# Autodesk Inventor assembly: A1-19027-400-06 Flange Comparison
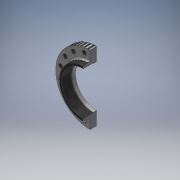
[picture p0: Inventor's stored thumbnail of the model, 180x180]
Saved by Autodesk Inventor 2017.3 (Build 213257000, 257)
## iProperties
Created: 2020-03-12
Part Number: A1-19027-400-06 Flange Comparison
Document SubType Name: Assembly
Designer: BEM
Author: BEM
## Documents named in this file (4)
- N:\A1 - Projects\A1-19\A1-19027--Syncrude Aurora HT2 spools - SP-237\A1-19027-400-06 Flange Comparison.iam
- N:\A1 - Projects\A1-19\A1-19027--Syncrude Aurora HT2 spools - SP-237\A1-19027-400-06 Alco flange - 12in CL300.ipt
- N:\Inventor\Content Center Files\R2017\en-US\ASME B16.5(10)\ASME B16.5 Flange Lapped - Class 300 12.ipt
- N:\Inventor\Content Center Files\R2017\en-US\ASME B16.5(41)\ASME B16.5 Flange Welding Neck - Class 300 12.ipt
## Components (3 placed, 3 different names)
1. A1-19027-400-06 Alco flange - 12in CL300:1 — Mate:1, Flush:1
2. ASME B16.5 Flange Lapped - Class 300 12:1 — Mate:1, Mate:2, Flush:2
3. ASME B16.5 Flange Welding Neck - Class 300 12:1 — Mate:2, Flush:1, Flush:2
## Relationships (4: Mate 2, Flush 2)
- Mate:1: A1-19027-400-06 Alco flange - 12in CL300:1 ↔ ASME B16.5 Flange Lapped - Class 300 12:1
- Mate:2: ASME B16.5 Flange Lapped - Class 300 12:1 ↔ ASME B16.5 Flange Welding Neck - Class 300 12:1
- Flush:1: A1-19027-400-06 Alco flange - 12in CL300:1 ↔ ASME B16.5 Flange Welding Neck - Class 300 12:1
- Flush:2: ASME B16.5 Flange Lapped - Class 300 12:1 ↔ ASME B16.5 Flange Welding Neck - Class 300 12:1
